# Autodesk Inventor assembly: COXA_UNIT_ASM
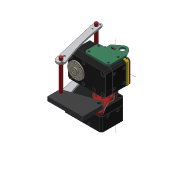
[picture p0: Inventor's stored thumbnail of the model, 180x180]
Saved by Autodesk Inventor 2019.4 (Build 234330000, 330)
## iProperties
Created: 2019-10-21
Part Number: COXA_UNIT_ASM
Material: 一般
Document SubType Name: Assembly
Designer: y6tada
Author: y6tada
## Documents named in this file (9)
- C:\Workspace\Yuni9\Inventor\Asm\COXA_UNIT\COXA_UNIT_ASM.iam
- C:\Workspace\Yuni9\Inventor\Libs\DYNAMIXEL\XM430\XM430_ASM_WITHOUT-BACK.iam
- C:\Workspace\Yuni9\Inventor\Asm\COXA_UNIT\COXA_YAW_SERVO_BASE.ipt
- C:\Workspace\Yuni9\Inventor\Asm\COXA_UNIT\COXA_YAW_SUPPORT-LINK_BACK.ipt
- C:\Workspace\Yuni9\Inventor\Asm\COXA_UNIT\COXA_ROLL_SERVO-OUTPUT.ipt
- C:\Workspace\Yuni9\Inventor\Asm\COXA_UNIT\COXA_ROLL_COUPLER_BACK.ipt
- C:\Workspace\Yuni9\Inventor\Asm\COXA_UNIT\COXA_YAW_BLOCK_ASM2.iam
- C:\Workspace\Yuni9\Inventor\Asm\COXA_UNIT\COXA_ROLL_LINK_ASM.iam
- C:\Workspace\Yuni9\Inventor\Asm\COXA_UNIT\COXA_YAW_SERVO_FRONT.ipt
## Components (8 placed, 8 different names)
1. COXA_YAW_SERVO_BASE:1 — フラッシュ:1, メイト:6, メイト:8, メイト:11, フラッシュ:4
2. XM430_ASM_WITHOUT-BACK:2 [sub-assembly] — メイト:7, メイト:23
3. COXA_YAW_SUPPORT-LINK_BACK:1 — メイト:8, メイト:11, メイト:13, メイト:25
4. COXA_ROLL_SERVO-OUTPUT:1 — メイト:12, メイト:13, メイト:17, メイト:23, メイト:25
5. COXA_ROLL_COUPLER_BACK:1 — メイト:17
6. COXA_YAW_BLOCK_ASM2:1 [sub-assembly] — メイト:27, フラッシュ:5
7. COXA_ROLL_LINK_ASM:1 [sub-assembly]
8. COXA_YAW_SERVO_FRONT:1 — フラッシュ:5
## Relationships (23: Mate 17, Flush 4, Angle 2)
- [Flush]: COXA_YAW_BLOCK_ASM2:1
- フラッシュ:1 [Flush]: COXA_YAW_SERVO_BASE:1
- メイト:6 [Mate]: COXA_YAW_SERVO_BASE:1
- 角度:1 [Angle] (0 deg)
- メイト:7 [Mate]: XM430_ASM_WITHOUT-BACK:2
- [Angle] (0 deg): XM430_ASM_WITHOUT-BACK:2 ↔ COXA_YAW_BLOCK_ASM2:1
- メイト:8 [Mate]: COXA_YAW_SERVO_BASE:1 ↔ COXA_YAW_SUPPORT-LINK_BACK:1
- メイト:11 [Mate] (0.3 mm): COXA_YAW_SERVO_BASE:1 ↔ COXA_YAW_SUPPORT-LINK_BACK:1
- メイト:12 [Mate]: COXA_ROLL_SERVO-OUTPUT:1
- メイト:13 [Mate]: COXA_YAW_SUPPORT-LINK_BACK:1 ↔ COXA_ROLL_SERVO-OUTPUT:1
- [Mate]: COXA_YAW_SUPPORT-LINK_BACK:1 ↔ COXA_ROLL_LINK_ASM:1
- [Mate] (0.5 mm): COXA_YAW_SUPPORT-LINK_BACK:1 ↔ COXA_ROLL_LINK_ASM:1
- メイト:17 [Mate]: COXA_ROLL_SERVO-OUTPUT:1 ↔ COXA_ROLL_COUPLER_BACK:1
- [Mate]: COXA_ROLL_COUPLER_BACK:1 ↔ COXA_ROLL_LINK_ASM:1
- [Mate]: COXA_YAW_SERVO_BASE:1 ↔ COXA_YAW_BLOCK_ASM2:1
- [Mate]: COXA_YAW_SERVO_BASE:1 ↔ COXA_YAW_BLOCK_ASM2:1
- [Mate]: COXA_YAW_SERVO_BASE:1 ↔ COXA_YAW_BLOCK_ASM2:1
- メイト:23 [Mate]: XM430_ASM_WITHOUT-BACK:2 ↔ COXA_ROLL_SERVO-OUTPUT:1
- メイト:25 [Mate] (0.3 mm): COXA_YAW_SUPPORT-LINK_BACK:1 ↔ COXA_ROLL_SERVO-OUTPUT:1
- [Mate]: COXA_ROLL_COUPLER_BACK:1 ↔ COXA_ROLL_LINK_ASM:1
- フラッシュ:4 [Flush]: COXA_YAW_SERVO_BASE:1
- メイト:27 [Mate]: COXA_YAW_BLOCK_ASM2:1
- フラッシュ:5 [Flush]: COXA_YAW_BLOCK_ASM2:1 ↔ COXA_YAW_SERVO_FRONT:1
